# Autodesk Inventor assembly: Pancake_Timing Assy_Star Shaft_3 Lanes
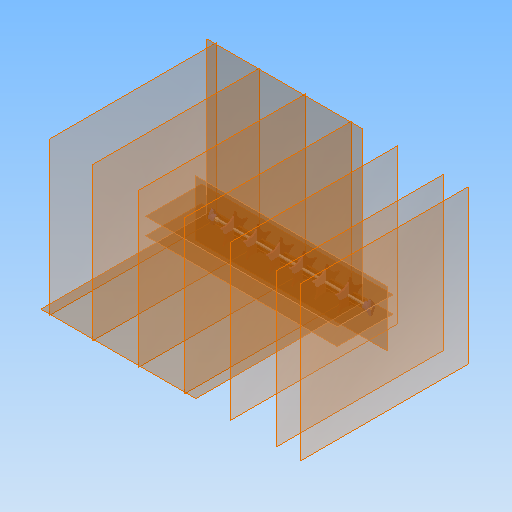
[picture p0: Inventor's stored thumbnail of the model, 512x512]
Saved by Autodesk Inventor 2018.1 (Build 221171000, 171)
## iProperties
Created: 2019-02-11
Part Number: Pancake_Timing Assy_Star Shaft_3 Lanes
Document SubType Name: Assembly
Designer: James
Mass: 92.827 g
Surface Area: 261.339 cm^2
Volume: 33.0472 cm^3
Density: 2.80892 g/cm^3
Author: James
## Documents named in this file (5)
- C:\Users\admin\Desktop\Ball-Machine\Pancake Sort\Pancake - 3 Lanes\Pancake_Timing Assy_Star Shaft_3 Lanes.iam
- C:\Users\admin\Desktop\Ball-Machine\Timing Gate\Timing_Star.ipt
- C:\Users\admin\Desktop\Ball-Machine\Prototype CAD\Selection Sort - 40mm\BS 3673 - 6mm External Circlip.ipt
- C:\Users\admin\Desktop\Ball-Machine\Prototype CAD\Selection Sort - 40mm\SAFL212 Oval 2 Bolt Flanged Unit.ipt
- C:\Users\admin\Desktop\Ball-Machine\Pancake Sort\Pancake - 3 Lanes\Pancake_Star Shaft_3 Lanes.ipt
## Components (17 placed, 4 different names)
1. Pancake_Star Shaft_3 Lanes:1 — Mate:4, Mate:49, Mate:50, Mate:61, Mate:62, Mate:63, Mate:66, Mate:68
2. SAFL212 Oval 2 Bolt Flanged Unit:1 — Mate:61, Flush:24, Angle:4, Mate:65
3. SAFL212 Oval 2 Bolt Flanged Unit:2 — Mate:62, Flush:24, Mate:64, Mate:67
4. BS 3673 - 6mm External Circlip:16 — Mate:65, Mate:66, Flush:25, Mate:68
5. BS 3673 - 6mm External Circlip:17 — Mate:63, Mate:64, Flush:25, Flush:26
6. BS 3673 - 6mm External Circlip:11 — Mate:49, Mate:50, Flush:26, Mate:69
7. Timing_Star:1 — Mate:4, Mate:69
8. BS 3673 - 6mm External Circlip:12
9. Timing_Star:2
10. BS 3673 - 6mm External Circlip:13
11. Timing_Star:3
12. BS 3673 - 6mm External Circlip:14
13. Timing_Star:4
14. BS 3673 - 6mm External Circlip:15
15. Timing_Star:5
16. BS 3673 - 6mm External Circlip:18
17. Timing_Star:6
## Component patterns: (6 elements, first: BS 3673 - 6mm External Circlip:11 + Timing_Star:1)
## Relationships (23: Mate 12, Flush 9, Angle 2)
- Mate:4: Pancake_Star Shaft_3 Lanes:1 ↔ Timing_Star:1
- [Flush]: Pancake_Star Shaft_3 Lanes:1
- Flush:11 (-58 mm)
- Flush:12 (-5 mm)
- Flush:13 (30 mm)
- [Flush]: Pancake_Star Shaft_3 Lanes:1
- [Flush]: Pancake_Star Shaft_3 Lanes:1
- Mate:49: Pancake_Star Shaft_3 Lanes:1 ↔ BS 3673 - 6mm External Circlip:11
- Mate:50: Pancake_Star Shaft_3 Lanes:1 ↔ BS 3673 - 6mm External Circlip:11
- [Angle] (0 deg): Pancake_Star Shaft_3 Lanes:1 ↔ BS 3673 - 6mm External Circlip:11
- Mate:61: Pancake_Star Shaft_3 Lanes:1 ↔ SAFL212 Oval 2 Bolt Flanged Unit:1
- Mate:62: Pancake_Star Shaft_3 Lanes:1 ↔ SAFL212 Oval 2 Bolt Flanged Unit:2
- Flush:24: SAFL212 Oval 2 Bolt Flanged Unit:1 ↔ SAFL212 Oval 2 Bolt Flanged Unit:2
- Angle:4 (0 deg): SAFL212 Oval 2 Bolt Flanged Unit:1
- Mate:63: Pancake_Star Shaft_3 Lanes:1 ↔ BS 3673 - 6mm External Circlip:17
- Mate:64: SAFL212 Oval 2 Bolt Flanged Unit:2 ↔ BS 3673 - 6mm External Circlip:17
- Mate:65: SAFL212 Oval 2 Bolt Flanged Unit:1 ↔ BS 3673 - 6mm External Circlip:16
- Mate:66: Pancake_Star Shaft_3 Lanes:1 ↔ BS 3673 - 6mm External Circlip:16
- Flush:25: BS 3673 - 6mm External Circlip:16 ↔ BS 3673 - 6mm External Circlip:17
- Flush:26: BS 3673 - 6mm External Circlip:17 ↔ BS 3673 - 6mm External Circlip:11
- Mate:67: SAFL212 Oval 2 Bolt Flanged Unit:2
- Mate:69: BS 3673 - 6mm External Circlip:11 ↔ Timing_Star:1
- Mate:68: Pancake_Star Shaft_3 Lanes:1 ↔ BS 3673 - 6mm External Circlip:16
